# Autodesk Inventor assembly: bridge_final
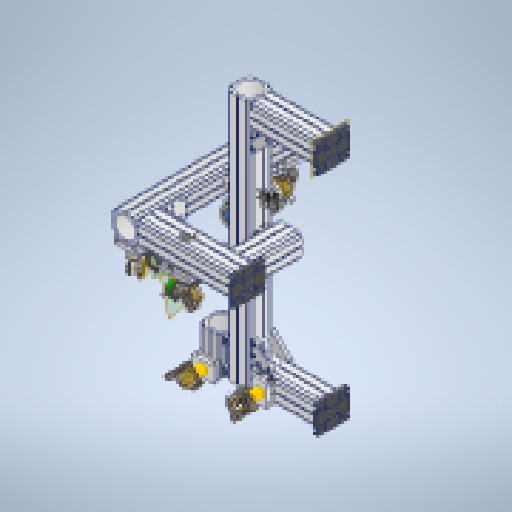
[picture p0: Inventor's stored thumbnail of the model, 512x512]
Saved by Autodesk Inventor 2026.1 (Build 301233000, 233)
## iProperties
Created: 2019-04-04
Part Number: bridge_final
Document SubType Name: Assembly
Designer: rainer
Author: rainer
## Documents named in this file (18)
- C:\Users\user\Desktop\setup for publishing\bridge_final.iam
- C:\Users\user\Desktop\setup for publishing\Thorlabs_66mm-rail_300mm.ipt
- C:\Users\user\Desktop\setup for publishing\XT66P1-66mm_mountin_bracket.ipt
- C:\Users\user\Desktop\setup for publishing\XT66RA1-66mm-angle-bracket.ipt
- C:\Users\user\Desktop\setup for publishing\Thorlabs_66mm-rail_700mm.ipt
- C:\Users\user\Desktop\setup for publishing\Thorlabs_66mm-rail_kurz.ipt
- C:\Users\user\Desktop\setup for publishing\XT66CC-cross-clamp.ipt
- C:\Users\user\Desktop\setup for publishing\XT66-rail_66_500.ipt
- C:\Users\user\Desktop\setup for publishing\66_100_rail+mount.iam
- C:\Users\user\Desktop\setup for publishing\Thorlabs_66mm-rail_359,672mm.ipt
- C:\Users\user\Desktop\setup for publishing\mirror_assembly_70mm.iam
- C:\Users\user\Desktop\setup for publishing\mirror_assembly_final - Kopie.iam
- C:\Users\user\Desktop\setup for publishing\mirror_assembly_final - Kopie (2).iam
- C:\Users\user\Desktop\setup for publishing\45deg_mirror_assembly.iam
- C:\Users\user\Desktop\setup for publishing\mirror_assembly_final.iam
- C:\Users\user\Desktop\setup for publishing\mirror_assembly_final - Kopie (3).iam
- C:\Users\user\Desktop\setup for publishing\NikkonTubelensBridge.iam
- C:\Users\user\Desktop\setup for publishing\SM1_LensBridge_160mm.iam
## Components (23 placed, 17 different names)
1. Thorlabs_66mm-rail_700mm:1 — Passend:1, Fluchtend:2, Passend:5, Passend:20, Passend:27, Fluchtend:47, Passend:53, Fluchtend:61, Passend:60, Fluchtend:70, Fluchtend:71, Passend:65, Fluchtend:75, Fluchtend:86, Fluchtend:92
2. Thorlabs_66mm-rail_300mm:1 — Passend:1, Fluchtend:2, Passend:3, Passend:6, Fluchtend:9, Fluchtend:86, Fluchtend:98, Fluchtend:99
3. Thorlabs_66mm-rail_300mm:3 — Passend:20, Passend:21, Fluchtend:23, Fluchtend:24, Fluchtend:47, Passend:76, Fluchtend:85, Passend:88, Passend:89, Fluchtend:92
4. Thorlabs_66mm-rail_359,672mm:1 — Passend:69, Fluchtend:80, Passend:70, Fluchtend:82, Fluchtend:83, Passend:71, Fluchtend:84, Passend:86, Passend:87, Fluchtend:97, Passend:107, Passend:108
5. Thorlabs_66mm-rail_kurz:4 — Passend:77, Passend:82
6. XT66-rail_66_500:1 — Fluchtend:63, Passend:54, Passend:70, Fluchtend:82, Fluchtend:83, Passend:72, Passend:90, Passend:91, Passend:94, Passend:95, Passend:102, Passend:103
7. 66_100_rail+mount:1 [sub-assembly] — Passend:60, Fluchtend:70, Fluchtend:71, Passend:96, Passend:97
8. XT66P1-66mm_mountin_bracket:1 — Passend:3, Fluchtend:79, Fluchtend:98, Fluchtend:99
9. XT66P1-66mm_mountin_bracket:3 — Passend:21, Fluchtend:23, Fluchtend:24, Fluchtend:93
10. XT66P1-66mm_mountin_bracket:4 — Passend:69, Fluchtend:80, Passend:98, Fluchtend:97
11. XT66RA1-66mm-angle-bracket:1 — Passend:5, Passend:6, Fluchtend:9
12. XT66RA1-66mm-angle-bracket:3 — Passend:27, Passend:76, Fluchtend:85
13. XT66RA1-66mm-angle-bracket:4 — Passend:71, Passend:72, Fluchtend:84
14. XT66CC-cross-clamp:3 — Passend:53, Fluchtend:61, Fluchtend:63, Passend:54
15. XT66CC-cross-clamp:4 — Passend:65, Fluchtend:75
16. 45deg_mirror_assembly:1 [sub-assembly] — Passend:86, Passend:87, Fluchtend:95, Passend:98
17. mirror_assembly_70mm:1 [sub-assembly] — Passend:77, Passend:82, Fluchtend:94, Passend:93
18. mirror_assembly_final - Kopie (3):1 [sub-assembly] — Passend:90, Passend:91, Fluchtend:94, Passend:104
19. mirror_assembly_final - Kopie (2):1 [sub-assembly] — Passend:94, Passend:95, Fluchtend:95, Passend:109
20. mirror_assembly_final - Kopie:1 [sub-assembly] — Passend:92, Passend:93, Passend:96, Passend:97
21. mirror_assembly_final:1 [sub-assembly] — Passend:88, Passend:89, Fluchtend:93, Passend:92
22. NikkonTubelensBridge:1 [sub-assembly] — Passend:102, Passend:103, Passend:104
23. SM1_LensBridge_160mm:1 [sub-assembly] — Passend:107, Passend:108, Passend:109
## Relationships (64: Mate 38, Flush 26)
- Passend:1 [Mate]: Thorlabs_66mm-rail_700mm:1 ↔ Thorlabs_66mm-rail_300mm:1
- Fluchtend:2 [Flush]: Thorlabs_66mm-rail_700mm:1 ↔ Thorlabs_66mm-rail_300mm:1
- Passend:3 [Mate]: Thorlabs_66mm-rail_300mm:1 ↔ XT66P1-66mm_mountin_bracket:1
- Passend:5 [Mate]: Thorlabs_66mm-rail_700mm:1 ↔ XT66RA1-66mm-angle-bracket:1
- Passend:6 [Mate]: Thorlabs_66mm-rail_300mm:1 ↔ XT66RA1-66mm-angle-bracket:1
- Fluchtend:9 [Flush] (1 mm): Thorlabs_66mm-rail_300mm:1 ↔ XT66RA1-66mm-angle-bracket:1
- Passend:20 [Mate]: Thorlabs_66mm-rail_700mm:1 ↔ Thorlabs_66mm-rail_300mm:3
- Passend:21 [Mate]: Thorlabs_66mm-rail_300mm:3 ↔ XT66P1-66mm_mountin_bracket:3
- Fluchtend:23 [Flush] (-5.08 mm): Thorlabs_66mm-rail_300mm:3 ↔ XT66P1-66mm_mountin_bracket:3
- Fluchtend:24 [Flush] (-11.621 mm): Thorlabs_66mm-rail_300mm:3 ↔ XT66P1-66mm_mountin_bracket:3
- Passend:27 [Mate]: Thorlabs_66mm-rail_700mm:1 ↔ XT66RA1-66mm-angle-bracket:3
- Fluchtend:47 [Flush]: Thorlabs_66mm-rail_700mm:1 ↔ Thorlabs_66mm-rail_300mm:3
- Passend:53 [Mate]: Thorlabs_66mm-rail_700mm:1 ↔ XT66CC-cross-clamp:3
- Fluchtend:61 [Flush]: Thorlabs_66mm-rail_700mm:1 ↔ XT66CC-cross-clamp:3
- Fluchtend:63 [Flush]: XT66-rail_66_500:1 ↔ XT66CC-cross-clamp:3
- Passend:54 [Mate]: XT66-rail_66_500:1 ↔ XT66CC-cross-clamp:3
- Passend:60 [Mate]: Thorlabs_66mm-rail_700mm:1 ↔ 66_100_rail+mount:1
- Fluchtend:70 [Flush]: Thorlabs_66mm-rail_700mm:1 ↔ 66_100_rail+mount:1
- Fluchtend:71 [Flush]: Thorlabs_66mm-rail_700mm:1 ↔ 66_100_rail+mount:1
- [Flush]: Thorlabs_66mm-rail_kurz:4 ↔ XT66CC-cross-clamp:4
- [Mate]: Thorlabs_66mm-rail_kurz:4 ↔ XT66CC-cross-clamp:4
- [Flush]: Thorlabs_66mm-rail_kurz:4 ↔ XT66CC-cross-clamp:4
- Passend:65 [Mate]: Thorlabs_66mm-rail_700mm:1 ↔ XT66CC-cross-clamp:4
- Fluchtend:75 [Flush]: Thorlabs_66mm-rail_700mm:1 ↔ XT66CC-cross-clamp:4
- Fluchtend:79 [Flush]: XT66P1-66mm_mountin_bracket:1
- Passend:69 [Mate]: Thorlabs_66mm-rail_359,672mm:1 ↔ XT66P1-66mm_mountin_bracket:4
- Fluchtend:80 [Flush] (-5.08 mm): Thorlabs_66mm-rail_359,672mm:1 ↔ XT66P1-66mm_mountin_bracket:4
- Passend:70 [Mate]: Thorlabs_66mm-rail_359,672mm:1 ↔ XT66-rail_66_500:1
- Fluchtend:82 [Flush]: Thorlabs_66mm-rail_359,672mm:1 ↔ XT66-rail_66_500:1
- Fluchtend:83 [Flush]: Thorlabs_66mm-rail_359,672mm:1 ↔ XT66-rail_66_500:1
- Passend:71 [Mate]: Thorlabs_66mm-rail_359,672mm:1 ↔ XT66RA1-66mm-angle-bracket:4
- Passend:72 [Mate]: XT66-rail_66_500:1 ↔ XT66RA1-66mm-angle-bracket:4
- Fluchtend:84 [Flush] (1 mm): Thorlabs_66mm-rail_359,672mm:1 ↔ XT66RA1-66mm-angle-bracket:4
- Passend:76 [Mate]: Thorlabs_66mm-rail_300mm:3 ↔ XT66RA1-66mm-angle-bracket:3
- Fluchtend:85 [Flush] (-1 mm): Thorlabs_66mm-rail_300mm:3 ↔ XT66RA1-66mm-angle-bracket:3
- Fluchtend:86 [Flush]: Thorlabs_66mm-rail_700mm:1 ↔ Thorlabs_66mm-rail_300mm:1
- Passend:77 [Mate]: Thorlabs_66mm-rail_kurz:4 ↔ mirror_assembly_70mm:1
- Passend:82 [Mate]: Thorlabs_66mm-rail_kurz:4 ↔ mirror_assembly_70mm:1
- Passend:86 [Mate]: Thorlabs_66mm-rail_359,672mm:1 ↔ 45deg_mirror_assembly:1
- Passend:87 [Mate]: Thorlabs_66mm-rail_359,672mm:1 ↔ 45deg_mirror_assembly:1
- Passend:88 [Mate]: Thorlabs_66mm-rail_300mm:3 ↔ mirror_assembly_final:1
- Passend:89 [Mate]: Thorlabs_66mm-rail_300mm:3 ↔ mirror_assembly_final:1
- Passend:90 [Mate]: XT66-rail_66_500:1 ↔ mirror_assembly_final - Kopie (3):1
- Passend:91 [Mate]: XT66-rail_66_500:1 ↔ mirror_assembly_final - Kopie (3):1
- Fluchtend:92 [Flush]: Thorlabs_66mm-rail_700mm:1 ↔ Thorlabs_66mm-rail_300mm:3
- Fluchtend:93 [Flush] (153.4 mm): XT66P1-66mm_mountin_bracket:3 ↔ mirror_assembly_final:1
- Passend:92 [Mate]: mirror_assembly_final - Kopie:1 ↔ mirror_assembly_final:1
- Fluchtend:94 [Flush]: mirror_assembly_70mm:1 ↔ mirror_assembly_final - Kopie (3):1
- Passend:93 [Mate]: mirror_assembly_70mm:1 ↔ mirror_assembly_final - Kopie:1
- Passend:94 [Mate]: XT66-rail_66_500:1 ↔ mirror_assembly_final - Kopie (2):1
- Passend:95 [Mate]: XT66-rail_66_500:1 ↔ mirror_assembly_final - Kopie (2):1
- Passend:96 [Mate]: 66_100_rail+mount:1 ↔ mirror_assembly_final - Kopie:1
- Passend:97 [Mate]: 66_100_rail+mount:1 ↔ mirror_assembly_final - Kopie:1
- Fluchtend:95 [Flush]: 45deg_mirror_assembly:1 ↔ mirror_assembly_final - Kopie (2):1
- Passend:98 [Mate] (-151.463 mm): XT66P1-66mm_mountin_bracket:4 ↔ 45deg_mirror_assembly:1
- Fluchtend:97 [Flush] (-11.621 mm): Thorlabs_66mm-rail_359,672mm:1 ↔ XT66P1-66mm_mountin_bracket:4
- Fluchtend:98 [Flush] (-5.08 mm): Thorlabs_66mm-rail_300mm:1 ↔ XT66P1-66mm_mountin_bracket:1
- Fluchtend:99 [Flush] (11.621 mm): Thorlabs_66mm-rail_300mm:1 ↔ XT66P1-66mm_mountin_bracket:1
- Passend:102 [Mate]: XT66-rail_66_500:1 ↔ NikkonTubelensBridge:1
- Passend:103 [Mate]: XT66-rail_66_500:1 ↔ NikkonTubelensBridge:1
- Passend:104 [Mate] (110 mm): mirror_assembly_final - Kopie (3):1 ↔ NikkonTubelensBridge:1
- Passend:107 [Mate]: Thorlabs_66mm-rail_359,672mm:1 ↔ SM1_LensBridge_160mm:1
- Passend:108 [Mate]: Thorlabs_66mm-rail_359,672mm:1 ↔ SM1_LensBridge_160mm:1
- Passend:109 [Mate] (90 mm): mirror_assembly_final - Kopie (2):1 ↔ SM1_LensBridge_160mm:1
## Named parameters: d172_d122_d66 = 0 mm, d173_d125_d110 = 0 mm, d174_d126_d111 = 0 mm
